# Autodesk Inventor assembly: Bearing Block Assem
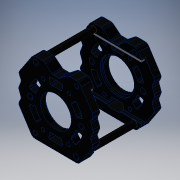
[picture p0: Inventor's stored thumbnail of the model, 180x180]
Saved by Autodesk Inventor 2019 (Build 230136000, 136)
## iProperties
Created: 2018-11-11
Part Number: Bearing Block Assem
Document SubType Name: Assembly
Designer: maste
Author: maste
## Documents named in this file (4)
- D:\Summer Drive Base V1\Summer Drivebase\Bearing Block Assem.iam
- D:\Summer Drive Base V1\Summer Drivebase\VersaBlock_Kit_217-3432.ipt
- D:\Summer Drive Base V1\Summer Drivebase\Ignore this-For constraining purposes.ipt
- D:\Summer Drive Base V1\Summer Drivebase\Pretend this is a bolt.ipt
## Components (6 placed, 3 different names)
1. VersaBlock_Kit_217-3432:1 — Mate:13, Mate:14, Mate:15, Mate:16, Rotation:1, Rotation:2, Mate:21, Mate:22, Mate:23
2. VersaBlock_Kit_217-3432:2 — Mate:4, Mate:5, Mate:6, Mate:17, Mate:18, Mate:19, Mate:20, Rotation:3, Rotation:4
3. Ignore this-For constraining purposes:3 — Mate:4, Mate:5, Mate:6
4. Pretend this is a bolt:1 — Mate:13, Mate:16, Rotation:1, Mate:17, Mate:20, Rotation:3
5. Pretend this is a bolt:2 — Mate:14, Mate:15, Rotation:2, Mate:18, Mate:19, Rotation:4
6. Ignore this-For constraining purposes:4 — Mate:21, Mate:22, Mate:23
## Relationships (18: Mate 14, RelateRotation 4)
- Mate:4: VersaBlock_Kit_217-3432:2 ↔ Ignore this-For constraining purposes:3
- Mate:5: VersaBlock_Kit_217-3432:2 ↔ Ignore this-For constraining purposes:3
- Mate:6: VersaBlock_Kit_217-3432:2 ↔ Ignore this-For constraining purposes:3
- Mate:13: VersaBlock_Kit_217-3432:1 ↔ Pretend this is a bolt:1
- Mate:14: VersaBlock_Kit_217-3432:1 ↔ Pretend this is a bolt:2
- Mate:15: VersaBlock_Kit_217-3432:1 ↔ Pretend this is a bolt:2
- Mate:16: VersaBlock_Kit_217-3432:1 ↔ Pretend this is a bolt:1
- Rotation:1 [RelateRotation] (1 ul): VersaBlock_Kit_217-3432:1 ↔ Pretend this is a bolt:1
- Rotation:2 [RelateRotation] (1 ul): VersaBlock_Kit_217-3432:1 ↔ Pretend this is a bolt:2
- Mate:17: VersaBlock_Kit_217-3432:2 ↔ Pretend this is a bolt:1
- Mate:18: VersaBlock_Kit_217-3432:2 ↔ Pretend this is a bolt:2
- Mate:19: VersaBlock_Kit_217-3432:2 ↔ Pretend this is a bolt:2
- Mate:20: VersaBlock_Kit_217-3432:2 ↔ Pretend this is a bolt:1
- Rotation:3 [RelateRotation] (1 ul): VersaBlock_Kit_217-3432:2 ↔ Pretend this is a bolt:1
- Rotation:4 [RelateRotation] (1 ul): VersaBlock_Kit_217-3432:2 ↔ Pretend this is a bolt:2
- Mate:21: VersaBlock_Kit_217-3432:1 ↔ Ignore this-For constraining purposes:4
- Mate:22: VersaBlock_Kit_217-3432:1 ↔ Ignore this-For constraining purposes:4
- Mate:23: VersaBlock_Kit_217-3432:1 ↔ Ignore this-For constraining purposes:4
